# Autodesk Inventor assembly: 10to1GearRatio
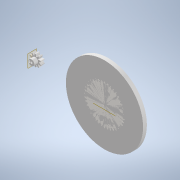
[picture p0: Inventor's stored thumbnail of the model, 180x180]
Saved by Autodesk Inventor 2020 (Build 240168000, 168)
## iProperties
Created: 2020-09-23
Part Number: 10to1GearRatio
Document SubType Name: Assembly
Designer: s4393944
Author: s4393944
## Documents named in this file (4)
- \\puffball.labs.eait.uq.edu.au\s4393944\Desktop\THESIS\CAD_MODEL\FINAL\turntable\Gears\10to1GearRatio.iam
- \\puffball.labs.eait.uq.edu.au\s4393944\Desktop\THESIS\CAD_MODEL\FINAL\turntable\Gears\Gear1.ipt
- \\puffball.labs.eait.uq.edu.au\s4393944\Desktop\THESIS\CAD_MODEL\FINAL\turntable\Gears\Gear2.ipt
- \\puffball.labs.eait.uq.edu.au\s4393944\Desktop\THESIS\CAD_MODEL\FINAL\turntable\Gears\4to1GearRatio\Design Accelerator\Spur Gears1.iam
## Components (3 placed, 3 different names)
1. Gear1:1 — Flush:1
2. Gear2:1 — Flush:1, Mate:1, Flush:2
3. Spur Gears:1 [sub-assembly] — Mate:1, Flush:2
## Relationships (3: Flush 2, Mate 1)
- Flush:1: Gear1:1 ↔ Gear2:1
- Mate:1: Gear2:1 ↔ Spur Gears:1
- Flush:2: Gear2:1 ↔ Spur Gears:1
